# Autodesk Inventor assembly: Guida a terra
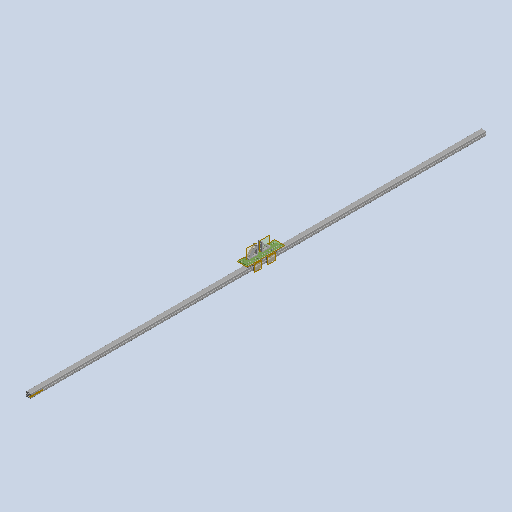
[picture p0: Inventor's stored thumbnail of the model, 512x512]
Saved by Autodesk Inventor 2022 (Build 260153000, 153)
## iProperties
RuleStatus: InUse
Part Number: Guida a terra
Document SubType Name: Assieme
Designer: matte
Author: matte
## Documents named in this file (3)
- C:\Users\Elia\Documents\ELIA\UNITN\MAGISTRALE\1st year\1st semester\Mechanical Design\Project\MDM-CyberOrto-CAD-main\Guida a terra.iam
- C:\Users\Elia\Documents\ELIA\UNITN\MAGISTRALE\1st year\1st semester\Mechanical Design\Project\MDM-CyberOrto-CAD-main\Pezzi singoli\Supporto lineare\Guida con supporto.iam
- C:\Users\Elia\Documents\ELIA\UNITN\MAGISTRALE\1st year\1st semester\Mechanical Design\Project\MDM-CyberOrto-CAD-main\Pezzi singoli\Pista Orizzontale.iam
## Components (2 placed, 2 different names)
1. Guida con supporto:1 [sub-assembly]
2. Pista Orizzontale:1 [sub-assembly]
## Relationships (5: Mate 5)
- [Mate]: Pista Orizzontale:1
- [Mate]: Pista Orizzontale:1
- [Mate]: Pista Orizzontale:1
- [Mate] (20 mm): Guida con supporto:1 ↔ Pista Orizzontale:1
- [Mate] (-40 mm): Guida con supporto:1 ↔ Pista Orizzontale:1
